# Autodesk Inventor assembly: Ensamblaje_final
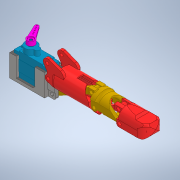
[picture p0: Inventor's stored thumbnail of the model, 180x180]
Saved by Autodesk Inventor 2020.4 (Build 244396010, 396A)
## iProperties
Created: 2021-11-02
Part Number: Ensamblaje_final
Document SubType Name: Assembly
Designer: chalo
Author: chalo
## Documents named in this file (8)
- C:\Users\chalo\OneDrive\Documents\GitHub\Interfaces-Biomedicas-2021\Gonzalo Palarea\Inventor\Ensamblaje_Final\Ensamblaje_final.iam
- C:\Users\chalo\OneDrive\Documents\GitHub\Interfaces-Biomedicas-2021\Gonzalo Palarea\Inventor\tipo2\Base_v2.ipt
- C:\Users\chalo\OneDrive\Documents\GitHub\Interfaces-Biomedicas-2021\Gonzalo Palarea\Inventor\servoconbrazo.iam
- C:\Users\chalo\OneDrive\Documents\GitHub\Interfaces-Biomedicas-2021\Gonzalo Palarea\Inventor\modificaciones prototipo 2\Metacarpo_mod2.ipt
- C:\Users\chalo\OneDrive\Documents\GitHub\Interfaces-Biomedicas-2021\Gonzalo Palarea\Inventor\tipo2\Falange proxima.ipt
- C:\Users\chalo\OneDrive\Documents\GitHub\Interfaces-Biomedicas-2021\Gonzalo Palarea\Inventor\tipo2\Falange_media_distal.ipt
- C:\Users\chalo\OneDrive\Documents\GitHub\Interfaces-Biomedicas-2021\Gonzalo Palarea\Inventor\Ensamblaje_Final\Palanca_metacarpo_proxima.ipt
- C:\Users\chalo\OneDrive\Documents\GitHub\Interfaces-Biomedicas-2021\Gonzalo Palarea\Inventor\Ensamblaje_Final\palanca_proxima_media.ipt
## Components (7 placed, 7 different names)
1. Base_v2:1 — Mate:1, Insert:1, Angle:1, Mate:2, Flush:1
2. servoconbrazo:1 [sub-assembly] — Mate:1, Insert:1, Angle:1
3. Metacarpo_mod2:1 — Insert:2, Angle:2, Mate:2
4. Falange proxima:1 — Insert:2, Angle:2, Angle:3, Insert:3
5. Falange_media_distal:1 — Angle:3, Insert:3
6. Palanca_metacarpo_proxima:1 — Flush:2
7. palanca_proxima_media:1 — Flush:3
## Relationships (11: Insert 3, Angle 3, Flush 3, Mate 2)
- Mate:1: Base_v2:1 ↔ servoconbrazo:1
- Insert:1: Base_v2:1 ↔ servoconbrazo:1
- Angle:1 (0 deg): Base_v2:1 ↔ servoconbrazo:1
- Insert:2 (0.154 mm): Metacarpo_mod2:1 ↔ Falange proxima:1
- Angle:2 (0 deg): Metacarpo_mod2:1 ↔ Falange proxima:1
- Angle:3 (0 deg): Falange proxima:1 ↔ Falange_media_distal:1
- Mate:2: Base_v2:1 ↔ Metacarpo_mod2:1
- Insert:3 (0.35 mm): Falange proxima:1 ↔ Falange_media_distal:1
- Flush:1 (2 mm): Base_v2:1
- Flush:2: Palanca_metacarpo_proxima:1
- Flush:3: palanca_proxima_media:1
